# Autodesk Inventor assembly: A2017_T2_10
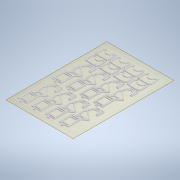
[picture p0: Inventor's stored thumbnail of the model, 180x180]
Saved by Autodesk Inventor 2020 (Build 240168000, 168)
## iProperties
Created: 2021-08-27
Part Number: A2017_T2_10
Document SubType Name: Assembly
Designer: Masato
Author: Masato
## Documents named in this file (4)
- C:\Inventor\SUSTAINA-OP\Cam\A2017_T2_10.iam
- C:\Inventor\SUSTAINA-OP\Cam\DisposableBoard.ipt
- C:\Inventor\SUSTAINA-OP\LowerBody\Ankle\Ankle_side_frame.ipt
- C:\Inventor\SUSTAINA-OP\LowerBody\Ankle\Ankle_back_frame.ipt
## Components (17 placed, 3 different names)
1. DisposableBoard:1 — メイト:2, メイト:1, フラッシュ:1, フラッシュ:2, メイト:5, フラッシュ:6, フラッシュ:8, メイト:6, フラッシュ:9
2. Ankle_back_frame:1 — メイト:6, メイト:7, フラッシュ:9
3. Ankle_back_frame:2
4. Ankle_back_frame:3
5. Ankle_back_frame:4
6. Ankle_back_frame:5
7. Ankle_back_frame:6
8. Ankle_back_frame:7
9. Ankle_back_frame:8
10. Ankle_side_frame:2 — メイト:5, フラッシュ:6, フラッシュ:8
11. Ankle_side_frame:3
12. Ankle_side_frame:4
13. Ankle_side_frame:5
14. Ankle_side_frame:6 — メイト:7
15. Ankle_side_frame:7
16. Ankle_side_frame:8
17. Ankle_side_frame:9
## Component patterns: (2 elements), (8 elements, first: Ankle_back_frame:1), (4 elements, first: Ankle_side_frame:2), コンポーネント パターン 12:2 (4 elements)
## Relationships (10: Mate 5, Flush 5)
- メイト:2 [Mate]: DisposableBoard:1
- メイト:1 [Mate]: DisposableBoard:1
- フラッシュ:1 [Flush]: DisposableBoard:1
- フラッシュ:2 [Flush]: DisposableBoard:1
- メイト:5 [Mate]: DisposableBoard:1 ↔ Ankle_side_frame:2
- フラッシュ:6 [Flush] (4 mm): DisposableBoard:1 ↔ Ankle_side_frame:2
- フラッシュ:8 [Flush] (2 mm): DisposableBoard:1 ↔ Ankle_side_frame:2
- メイト:6 [Mate]: DisposableBoard:1 ↔ Ankle_back_frame:1
- メイト:7 [Mate] (2.5 mm): Ankle_back_frame:1 ↔ Ankle_side_frame:6
- フラッシュ:9 [Flush] (4 mm): DisposableBoard:1 ↔ Ankle_back_frame:1
